# Autodesk Inventor assembly: Assembly1
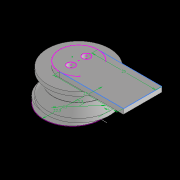
[picture p0: Inventor's stored thumbnail of the model, 180x180]
Saved by Autodesk Inventor 2022.2 (Build 262287010, 287A)
## iProperties
Created: 2022-06-03
Part Number: Assembly1
Document SubType Name: Assembly
Designer: Árni Þór Þorgeirsson
Author: Árni Þór Þorgeirsson
## Documents named in this file (4)
- G:\My Drive\Masters Thesis - exo\CAD_Files\External Hardware\Assembly1.iam
- G:\My Drive\Masters Thesis - exo\CAD_Files\ExoskeletonV0p2\Rotor_TSB\Axl.ipt
- G:\My Drive\Masters Thesis - exo\CAD_Files\ExoskeletonV0p2\Rotor_TSB\Leaver.ipt
- G:\My Drive\Masters Thesis - exo\CAD_Files\ExoskeletonV0p2\Rotor_TSB\Rotor_TSB.ipt
## Components (3 placed, 3 different names)
1. Axl:1 — Mate:1, Insert:1, Insert:2, Insert:3
2. Leaver:1 — Insert:2, Insert:3
3. Rotor_TSB:1 — Mate:1, Insert:1
## Relationships (4: Insert 3, Mate 1)
- Mate:1: Axl:1 ↔ Rotor_TSB:1
- Insert:1: Axl:1 ↔ Rotor_TSB:1
- Insert:2: Axl:1 ↔ Leaver:1
- Insert:3: Axl:1 ↔ Leaver:1
